# Autodesk Inventor assembly: Lifting Mechanism
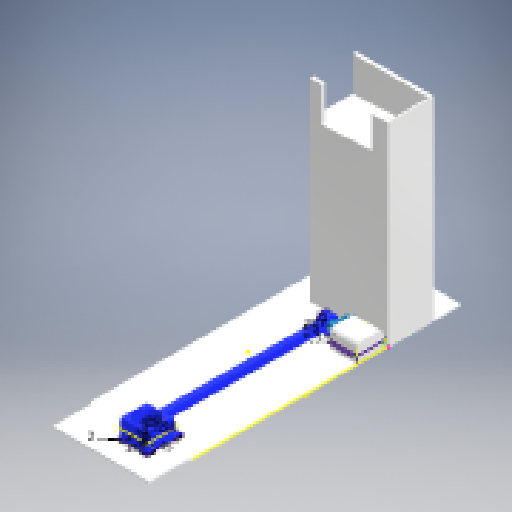
[picture p0: Inventor's stored thumbnail of the model, 512x512]
Saved by Autodesk Inventor 2025.3 (Build 293356000, 356)
## iProperties
Created: 2026-03-10
Part Number: Lifting Mechanism
Document SubType Name: Assembly
Designer: user
Author: user
## Documents named in this file (7)
- C:\Ayman\Inventor Projects\Lifting Mechanism\Lifting Mechanism.iam
- C:\Ayman\Inventor Projects\Lifting Mechanism\lifting base.ipt
- C:\Ayman\Inventor Projects\Lifting Mechanism\SERVO.ipt
- C:\Ayman\Inventor Projects\Lifting Mechanism\arm.ipt
- C:\Ayman\Inventor Projects\Lifting Mechanism\final sensor housing.ipt
- C:\Ayman\Inventor Projects\Lifting Mechanism\IR Module.ipt
- C:\Users\user\Documents\Inventor\Content Center Files\R2025\en-US\ISO 1207(3)\ISO 1207 - M3 x 5NF EN ISO.ipt
## Components (9 placed, 6 different names)
1. lifting base:1 — Mate:1, Mate:2, Mate:5
2. SERVO:1 — Mate:1, Mate:2, Mate:5, Mate:6, Mate:7
3. arm:2 — Mate:6, Mate:7, Mate:11, Mate:12, Mate:13, Mate:14, Mate:15, Mate:20, Mate:22
4. final sensor housing:1 — Mate:8, Mate:9, Mate:10, Mate:11, Mate:12, Mate:13, Mate:14, Mate:15, Mate:16, Mate:17, Mate:18, Mate:19, Mate:21, Mate:23
5. IR Module:1 — Mate:8, Mate:9, Mate:10
6. NF EN ISO 1207 M3 x 5:1 — Mate:16, Mate:17
7. NF EN ISO 1207 M3 x 5:2 — Mate:18, Mate:19
8. NF EN ISO 1207 M3 x 5:3 — Mate:20, Mate:21
9. NF EN ISO 1207 M3 x 5:4 — Mate:22, Mate:23
## Relationships (21: Mate 21)
- Mate:1: lifting base:1 ↔ SERVO:1
- Mate:2: lifting base:1 ↔ SERVO:1
- Mate:5: lifting base:1 ↔ SERVO:1
- Mate:6: SERVO:1 ↔ arm:2
- Mate:7: SERVO:1 ↔ arm:2
- Mate:8: final sensor housing:1 ↔ IR Module:1
- Mate:9: final sensor housing:1 ↔ IR Module:1
- Mate:10: final sensor housing:1 ↔ IR Module:1
- Mate:11: arm:2 ↔ final sensor housing:1
- Mate:12: arm:2 ↔ final sensor housing:1
- Mate:13: arm:2 ↔ final sensor housing:1
- Mate:14: arm:2 ↔ final sensor housing:1
- Mate:15: arm:2 ↔ final sensor housing:1
- Mate:16: final sensor housing:1 ↔ NF EN ISO 1207 M3 x 5:1
- Mate:17: final sensor housing:1 ↔ NF EN ISO 1207 M3 x 5:1
- Mate:18: final sensor housing:1 ↔ NF EN ISO 1207 M3 x 5:2
- Mate:19: final sensor housing:1 ↔ NF EN ISO 1207 M3 x 5:2
- Mate:20: arm:2 ↔ NF EN ISO 1207 M3 x 5:3
- Mate:21: final sensor housing:1 ↔ NF EN ISO 1207 M3 x 5:3
- Mate:22: arm:2 ↔ NF EN ISO 1207 M3 x 5:4
- Mate:23: final sensor housing:1 ↔ NF EN ISO 1207 M3 x 5:4
## Named parameters: Finish1_Area = 13.1132
note: some values were not read from the file. Shown as the stored number, unit unknown: "Finish1_Area".
